# Autodesk Inventor assembly: Xtra Cook
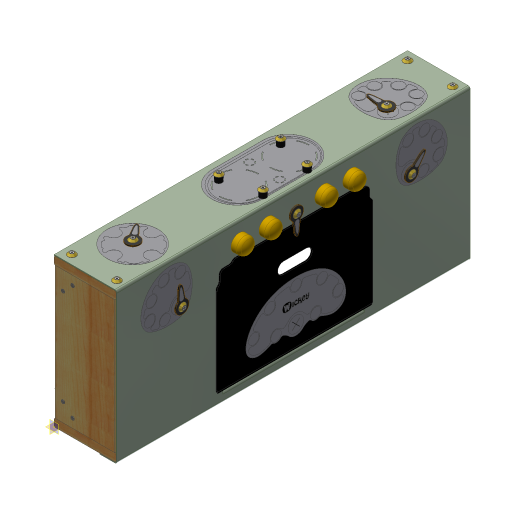
[picture p0: Inventor's stored thumbnail of the model, 512x512]
Saved by Autodesk Inventor 2024 (Build 280153000, 153)
## iProperties
Created: 2025-01-31
Part Number: Xtra Cook
Document SubType Name: Assembly
Designer: r.orschler
Assembly Measurements: /
Assembly Norm: /
Color: /
General Measurements: /
Packaging Manual: /
Packaging Method: /
Production Method: /
Tolerance: /
Weight: /
Author: r.orschler
## Documents named in this file (3)
- Z:\Entwicklung\INVENTOR\INVENTOR 2023\1 Products\Add Ons\Xtra Cook\Xtra Cook.iam
- Z:\Entwicklung\INVENTOR\INVENTOR 2023\2 Modules\14 Extra\Extra 071\Extra 071.iam
- Z:\Entwicklung\INVENTOR\INVENTOR 2023\2 Modules\15 Decoration\Decoration 209\Decoration 209.iam
## Components (2 placed, 2 different names)
1. Extra 071:1 [sub-assembly] — Mate:1, Mate:2, Mate:3, Mate:26
2. Decoration 209:1 [sub-assembly] — Mate:26
## Relationships (4: Mate 4)
- Mate:1: Extra 071:1
- Mate:2: Extra 071:1
- Mate:3: Extra 071:1
- Mate:26: Extra 071:1 ↔ Decoration 209:1
